# Autodesk Inventor assembly: Assembly2
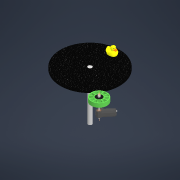
[picture p0: Inventor's stored thumbnail of the model, 180x180]
Saved by Autodesk Inventor 2022 (Build 260153000, 153)
## iProperties
Created: 2021-10-09
Part Number: Assembly2
Document SubType Name: Assembly
Designer: zehrab
Author: zehrab
## Documents named in this file (8)
- C:\Users\zehrab\Documents\Inventor\Duck Carousel\Assembly2.iam
- C:\Users\zehrab\Documents\Inventor\Duck Carousel\Carousel Base.ipt
- C:\Users\zehrab\Documents\Inventor\Duck Carousel\Carousel.ipt
- C:\Users\zehrab\Documents\Inventor\Duck Carousel\am-4510 Rubber Duck.ipt
- C:\Users\zehrab\Documents\Inventor\Duck Carousel\wheel.iam
- C:\Users\zehrab\Documents\Inventor\Duck Carousel\REV-41-1300.ipt
- C:\Users\zehrab\Documents\Inventor\Duck Carousel\REV-41-1349.ipt
- C:\Users\zehrab\Documents\Inventor\Duck Carousel\REV-21-1844.ipt
## Components (7 placed, 7 different names)
1. Carousel Base:1 — Mate:1, Flush:1
2. Carousel:1 — Mate:1, Flush:1, Mate:2, Tangent:1, Flush:2, Rotation:1
3. am-4510 Rubber Duck:1 — Mate:2
4. wheel:1 [sub-assembly] — Tangent:1, Flush:2, Rotation:1, Mate:3, Angle:2, Angle:3, Mate:4, Mate:5
5. REV-41-1300:1 — Angle:5, Mate:6, Mate:7
6. REV-41-1349:1 — Angle:4, Mate:5, Angle:5, Mate:6, Mate:7
7. REV-21-1844:1 — Mate:3, Angle:2, Angle:3, Mate:4, Angle:4
## Relationships (15: Mate 7, Angle 4, Flush 2, Tangent 1, RelateRotation 1)
- Mate:1: Carousel Base:1 ↔ Carousel:1
- Flush:1: Carousel Base:1 ↔ Carousel:1
- Mate:2: Carousel:1 ↔ am-4510 Rubber Duck:1
- Tangent:1: Carousel:1 ↔ wheel:1
- Flush:2: Carousel:1 ↔ wheel:1
- Rotation:1 [RelateRotation] (100 ul): Carousel:1 ↔ wheel:1
- Mate:3: wheel:1 ↔ REV-21-1844:1
- Angle:2 (0 deg): wheel:1 ↔ REV-21-1844:1
- Angle:3 (0 deg): wheel:1 ↔ REV-21-1844:1
- Mate:4: wheel:1 ↔ REV-21-1844:1
- Angle:4 (0 deg): REV-41-1349:1 ↔ REV-21-1844:1
- Mate:5: wheel:1 ↔ REV-41-1349:1
- Angle:5 (0 deg): REV-41-1300:1 ↔ REV-41-1349:1
- Mate:6: REV-41-1300:1 ↔ REV-41-1349:1
- Mate:7: REV-41-1300:1 ↔ REV-41-1349:1
